# Autodesk Inventor assembly: タミヤダンパーフロント56,74.6_MIR
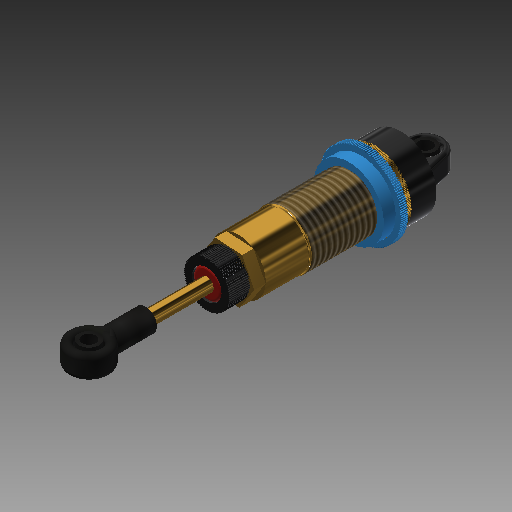
[picture p0: Inventor's stored thumbnail of the model, 512x512]
Saved by Autodesk Inventor 2019.2 (Build 232265000, 265)
## iProperties
Part Number: タミヤダンパーフロント56,74.6_MIR
Material: 一般
Document SubType Name: Assembly
Designer: 雪村
Mass: 29.9788 g
Surface Area: 59.981 cm^2
Volume: 5.28575 cm^3
Density: 5.67163 g/cm^3
Author: 雪村
## Documents named in this file (9)
- C:\Users\white\Documents\SRDC\SRDC\Inventor_2017\2018年機体\パーツ\タミヤダンパーフロント56,74.6_MIR.iam
- C:\Users\white\Documents\SRDC\SRDC\Inventor_2017\2018年機体\パーツ\タミヤダンパー2_MIR.ipt
- C:\Users\white\Documents\SRDC\SRDC\Inventor_2017\2018年機体\パーツ\タミヤダンパー3_MIR.ipt
- C:\Users\white\Documents\SRDC\SRDC\Inventor_2017\2018年機体\パーツ\タミヤダンパー4_MIR.ipt
- C:\Users\white\Documents\SRDC\SRDC\Inventor_2017\2018年機体\パーツ\タミヤダンパー5_MIR.ipt
- C:\Users\white\Documents\SRDC\SRDC\Inventor_2017\2018年機体\パーツ\タミヤダンパー7_MIR.ipt
- C:\Users\white\Documents\SRDC\SRDC\Inventor_2017\2018年機体\パーツ\タミヤダンパー6_MIR.ipt
- C:\Users\white\Documents\SRDC\SRDC\Inventor_2017\2018年機体\パーツ\タミヤダンパー8_MIR.ipt
- C:\Users\white\Documents\SRDC\SRDC\Inventor_2017\2018年機体\パーツ\タミヤダンパー9_MIR.ipt
## Components (9 placed, 8 different names)
1. タミヤダンパー2_MIR:1 — 挿入:1, フラッシュ:1, フラッシュ:3, ボール:2
2. タミヤダンパー3_MIR:1 — 挿入:1, 挿入:4, メイト:1
3. タミヤダンパー4_MIR:1 — 挿入:4, 挿入:3
4. タミヤダンパー5_MIR:1 — メイト:1
5. タミヤダンパー7_MIR:1 — 挿入:3
6. タミヤダンパー6_MIR:1 — 挿入:5
7. タミヤダンパー8_MIR:1 — 挿入:5, フラッシュ:1
8. タミヤダンパー9_MIR:1 — フラッシュ:3, フラッシュ:2, ボール:2
9. タミヤダンパー9_MIR:2 — フラッシュ:2
## Relationships (9: Insert 4, Flush 3, Mate 1, BallJoint 1)
- 挿入:1 [Insert]: タミヤダンパー2_MIR:1 ↔ タミヤダンパー3_MIR:1
- 挿入:4 [Insert]: タミヤダンパー3_MIR:1 ↔ タミヤダンパー4_MIR:1
- メイト:1 [Mate]: タミヤダンパー3_MIR:1 ↔ タミヤダンパー5_MIR:1
- 挿入:3 [Insert]: タミヤダンパー4_MIR:1 ↔ タミヤダンパー7_MIR:1
- 挿入:5 [Insert]: タミヤダンパー6_MIR:1 ↔ タミヤダンパー8_MIR:1
- フラッシュ:1 [Flush]: タミヤダンパー2_MIR:1 ↔ タミヤダンパー8_MIR:1
- フラッシュ:3 [Flush]: タミヤダンパー2_MIR:1 ↔ タミヤダンパー9_MIR:1
- フラッシュ:2 [Flush]: タミヤダンパー9_MIR:1 ↔ タミヤダンパー9_MIR:2
- ボール:2 [BallJoint]: タミヤダンパー2_MIR:1 ↔ タミヤダンパー9_MIR:1
